# Autodesk Inventor assembly: ensamble_general
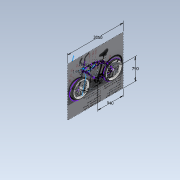
[picture p0: Inventor's stored thumbnail of the model, 180x180]
Saved by Autodesk Inventor 2021 (Build 250183000, 183)
## iProperties
Created: 2021-04-10
Part Number: ensamble_general
Document SubType Name: Assembly
Designer: j2seb
Author: j2seb
## Documents named in this file (4)
- C:\Git\Proyecto_APM\02 Inventor\ensamble_general.iam
- C:\Git\Proyecto_APM\02 Inventor\Marco_Bicicleta.iam
- C:\Git\Proyecto_APM\02 Inventor\Manubrio.ipt
- C:\Git\Proyecto_APM\02 Inventor\Ensamble_Llanta.iam
## Components (4 placed, 3 different names)
1. Marco_Bicicleta:1 [sub-assembly] — Coincidencia:1
2. Manubrio:1 — Coincidencia:1
3. Ensamble_Llanta:1 [sub-assembly]
4. Ensamble_Llanta:2 [sub-assembly]
## Relationships (1: Mate 1)
- Coincidencia:1 [Mate]: Marco_Bicicleta:1 ↔ Manubrio:1
